# Autodesk Inventor assembly: Tensionador-4-Cabos_Modelo2
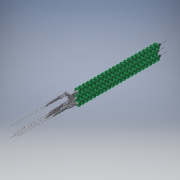
[picture p0: Inventor's stored thumbnail of the model, 180x180]
Saved by Autodesk Inventor 2018 (Build 220112000, 112)
## iProperties
Created: 2021-08-09
Part Number: Tensionador-4-Cabos_Modelo2
Document SubType Name: Assembly
Designer: L08619
Author: L08619
## Documents named in this file (6)
- F:\Projetos\TAESA\Modelo 3D - Tensionadores e Suspensão\Tensionador\Tensionador-4-Cabos_Modelo2.iam
- F:\Projetos\TAESA\Modelo 3D - Tensionadores e Suspensão\Tensionador\Balancim_4-Cabos_Modelo2.ipt
- F:\Projetos\TAESA\Modelo 3D - Tensionadores e Suspensão\Tensionador\Clevis-Socket.iam
- F:\Projetos\TAESA\Modelo 3D - Tensionadores e Suspensão\Tensionador\gpghmb32.iam
- F:\Projetos\TAESA\Modelo 3D - Tensionadores e Suspensão\Tensionador\SVEID single tension set.iam
- F:\Projetos\TAESA\Modelo 3D - Tensionadores e Suspensão\Suporte de Suspenção\Suspensao.ipt
## Components (19 placed, 5 different names)
1. Balancim_4-Cabos_Modelo2:1 — Mate:1, Flush:1, Cylindrical:1, Cylindrical:2, Cylindrical:3, Cylindrical:4, Cylindrical:5, Cylindrical:6, Cylindrical:7, Mate:2, Mate:3, Mate:4
2. Clevis-Socket:1 [sub-assembly] — Cylindrical:3, Mate:4, Cylindrical:12
3. Clevis-Socket:2 [sub-assembly] — Cylindrical:2, Mate:3, Rigid:1
4. Clevis-Socket:3 [sub-assembly] — Cylindrical:1, Mate:2, Cylindrical:11
5. gpghmb32:1 [sub-assembly] — Cylindrical:4
6. gpghmb32:3 [sub-assembly] — Cylindrical:5
7. gpghmb32:4 [sub-assembly] — Cylindrical:6
8. gpghmb32:5 [sub-assembly] — Cylindrical:7
9. SVEID single tension set:1 [sub-assembly] — Rotational:1
10. SVEID single tension set:2 [sub-assembly] — Cylindrical:8
11. SVEID single tension set:3 [sub-assembly] — Cylindrical:9
12. SVEID single tension set:5 [sub-assembly] — Cylindrical:10
13. gpghmb32:6 [sub-assembly] — Rotational:1
14. gpghmb32:7 [sub-assembly] — Cylindrical:8
15. gpghmb32:8 [sub-assembly] — Cylindrical:10
16. gpghmb32:9 [sub-assembly] — Cylindrical:9
17. Suspensao:1 — Cylindrical:12
18. Suspensao:2 — Cylindrical:11
19. Suspensao:3 — Rigid:1
## Relationships (19: CylindricalJoint 12, Mate 4, Flush 1, RevoluteJoint 1, WeldJoint 1)
- Mate:1: Balancim_4-Cabos_Modelo2:1
- Flush:1: Balancim_4-Cabos_Modelo2:1
- Cylindrical:1: Balancim_4-Cabos_Modelo2:1 ↔ Clevis-Socket:3
- Cylindrical:2: Balancim_4-Cabos_Modelo2:1 ↔ Clevis-Socket:2
- Cylindrical:3: Balancim_4-Cabos_Modelo2:1 ↔ Clevis-Socket:1
- Cylindrical:4: Balancim_4-Cabos_Modelo2:1 ↔ gpghmb32:1
- Cylindrical:5: Balancim_4-Cabos_Modelo2:1 ↔ gpghmb32:3
- Cylindrical:6: Balancim_4-Cabos_Modelo2:1 ↔ gpghmb32:4
- Cylindrical:7: Balancim_4-Cabos_Modelo2:1 ↔ gpghmb32:5
- Rotational:1 [RevoluteJoint]: SVEID single tension set:1 ↔ gpghmb32:6
- Cylindrical:8: SVEID single tension set:2 ↔ gpghmb32:7
- Cylindrical:9: SVEID single tension set:3 ↔ gpghmb32:9
- Cylindrical:10: SVEID single tension set:5 ↔ gpghmb32:8
- Mate:2 (2 mm): Balancim_4-Cabos_Modelo2:1 ↔ Clevis-Socket:3
- Mate:3 (2 mm): Balancim_4-Cabos_Modelo2:1 ↔ Clevis-Socket:2
- Mate:4 (2 mm): Balancim_4-Cabos_Modelo2:1 ↔ Clevis-Socket:1
- Cylindrical:11: Clevis-Socket:3 ↔ Suspensao:2
- Rigid:1 [WeldJoint]: Clevis-Socket:2 ↔ Suspensao:3
- Cylindrical:12: Clevis-Socket:1 ↔ Suspensao:1
